# Autodesk Inventor assembly: element
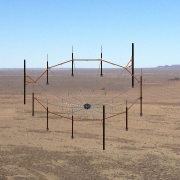
[picture p0: Inventor's stored thumbnail of the model, 180x180]
Saved by Autodesk Inventor 2013 SP2 (Build 170200200, 200)
## iProperties
Created: 2014-02-25
Part Number: element
Document SubType Name: Assembly
Designer: Dave
Author: Dave
## Documents named in this file (8)
- C:\Users\Dave\Desktop\hera-cad\element.iam
- C:\Users\Dave\Desktop\hera-cad\plat.ipt
- C:\Users\Dave\Desktop\hera-cad\support\poleAssembly.iam
- C:\Users\Dave\Desktop\hera-cad\support\postAssembly.iam
- C:\Users\Dave\Desktop\hera-cad\hub\hub.iam
- C:\Users\Dave\Desktop\hera-cad\surface\sparFull.ipt
- C:\Users\Dave\Desktop\hera-cad\support\sparAssembly.iam
- C:\Users\Dave\Desktop\hera-cad\support\rimAssembly.iam
## Components (50 placed, 7 different names)
1. plat:1 — Insert:1, Insert:3, Insert:4, Insert:5, Insert:6, Insert:7, Insert:8
2. poleAssembly:1 [sub-assembly] — Insert:1
3. poleAssembly:2 [sub-assembly] — Insert:4
4. poleAssembly:3 [sub-assembly] — Insert:3, Mate:1
5. hub:1 [sub-assembly] — Insert:8, Insert:9, Insert:10
6. postAssembly:3 [sub-assembly] — Insert:5
7. postAssembly:2 [sub-assembly] — Insert:6
8. postAssembly:1 [sub-assembly] — Insert:7
9. postAssembly:4 [sub-assembly]
10. postAssembly:5 [sub-assembly]
11. postAssembly:6 [sub-assembly]
12. postAssembly:7 [sub-assembly]
13. postAssembly:8 [sub-assembly]
14. postAssembly:9 [sub-assembly]
15. sparFull:1 — Insert:9
16. sparFull:2
17. sparFull:3
18. sparFull:4
19. sparFull:5
20. sparFull:6
21. sparFull:7
22. sparFull:8
23. sparFull:9
24. sparFull:10
25. sparFull:11
26. sparFull:12
27. rimAssembly:1 [sub-assembly] — Mate:1
28. rimAssembly:2 [sub-assembly]
29. rimAssembly:3 [sub-assembly]
30. rimAssembly:4 [sub-assembly]
31. rimAssembly:5 [sub-assembly]
32. rimAssembly:6 [sub-assembly]
33. rimAssembly:7 [sub-assembly]
34. rimAssembly:8 [sub-assembly]
35. rimAssembly:9 [sub-assembly]
36. rimAssembly:10 [sub-assembly]
37. rimAssembly:11 [sub-assembly]
38. rimAssembly:12 [sub-assembly]
39. sparAssembly:1 [sub-assembly] — Insert:10
40. sparAssembly:2 [sub-assembly]
41. sparAssembly:3 [sub-assembly]
42. sparAssembly:4 [sub-assembly]
43. sparAssembly:5 [sub-assembly]
44. sparAssembly:6 [sub-assembly]
45. sparAssembly:7 [sub-assembly]
46. sparAssembly:8 [sub-assembly]
47. sparAssembly:9 [sub-assembly]
48. sparAssembly:10 [sub-assembly]
49. sparAssembly:11 [sub-assembly]
50. sparAssembly:12 [sub-assembly]
## Component patterns: posts (3 elements), spars (12 elements), rim (12 elements), supportSpars (12 elements)
## Relationships (10: Insert 9, Mate 1)
- Insert:1 (-1000 mm): plat:1 ↔ poleAssembly:1
- Insert:3 (-1000 mm): plat:1 ↔ poleAssembly:3
- Insert:4 (-1000 mm): plat:1 ↔ poleAssembly:2
- Insert:5: plat:1 ↔ postAssembly:3
- Insert:6: plat:1 ↔ postAssembly:2
- Insert:7: plat:1 ↔ postAssembly:1
- Insert:8: plat:1 ↔ hub:1
- Insert:9 (-228.6 mm): hub:1 ↔ sparFull:1
- Insert:10 (-228.6 mm): hub:1 ↔ sparAssembly:1
- Mate:1: poleAssembly:3 ↔ rimAssembly:1
